# Autodesk Inventor assembly: Gripper V 10.0 assembly
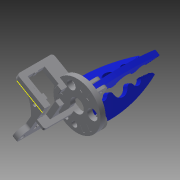
[picture p0: Inventor's stored thumbnail of the model, 180x180]
Saved by Autodesk Inventor 2015 (Build 190159000, 159)
## iProperties
Created: 2015-06-30
Part Number: Gripper V 10.0 assembly
Document SubType Name: Assembly
Designer: Stackpole
Author: Stackpole
## Documents named in this file (8)
- C:\Users\Stackpole\Desktop\Patrick!\Gripper Folder\Gripper V 10.0\Gripper V 10.0 assembly.iam
- C:\Users\Stackpole\Desktop\Patrick!\Gripper Folder\Gripper V 10.0\Gripper V 10.0 base 6mm.ipt
- C:\Users\Stackpole\Desktop\Patrick!\Gripper Folder\Gripper V 10.0\Gripper V 10.0 servo bracket right 6mm.ipt
- C:\Users\Stackpole\Desktop\Patrick!\Gripper Folder\Gripper V 10.0\Gripper V 10.1 servo bracket bottom 6mm.ipt
- C:\Users\Stackpole\Desktop\Patrick!\Gripper Folder\Gripper V 10.0\Gripper V 10.0 servo bracket side left 3mm.ipt
- C:\Users\Stackpole\Desktop\Patrick!\Gripper Folder\Gripper V 10.0\Gripper V 10.0 servo triangle bracket 3mm.ipt
- C:\Users\Stackpole\Desktop\Patrick!\Gripper Folder\Gripper V 10.0\Gripper V 10.0 base tab 3mm.ipt
- C:\Users\Stackpole\Desktop\Patrick!\Gripper Folder\Gripper V 10.0\Gripper V 10.0 finger master 6mm.ipt
## Components (14 placed, 7 different names)
1. Gripper V 10.0 base 6mm:1 — Mate:1, Mate:2, Mate:3, Mate:4, Mate:5, Mate:6, Mate:7, Mate:8, Mate:9, Mate:13, Mate:14, Mate:15, Mate:16, Mate:17, Mate:18, Mate:19, Mate:20, Mate:21, Mate:22, Mate:23, Mate:24, Mate:25, Mate:26, Mate:27, Mate:28, Mate:29, Mate:30, Mate:31
2. Gripper V 10.0 servo bracket right 6mm:1 — Mate:1, Mate:2, Mate:3, Mate:11
3. Gripper V 10.1 servo bracket bottom 6mm:1 — Mate:4, Mate:5, Mate:6, Mate:10, Mate:12
4. Gripper V 10.0 servo bracket side left 3mm:1 — Mate:7, Mate:8, Mate:9
5. Gripper V 10.0 servo triangle bracket 3mm:1 — Mate:10, Mate:11, Mate:12
6. Gripper V 10.0 finger master 6mm:1 — Insert:2
7. Gripper V 10.0 finger master 6mm:2 — Insert:3
8. Gripper V 10.0 finger master 6mm:3 — Insert:1
9. Gripper V 10.0 base tab 3mm:3 — Mate:13, Mate:22, Mate:27
10. Gripper V 10.0 base tab 3mm:4 — Mate:16, Mate:19, Mate:24, Mate:29
11. Gripper V 10.0 base tab 3mm:5 — Mate:17, Mate:20, Mate:31
12. Gripper V 10.0 base tab 3mm:6 — Mate:15, Mate:21, Mate:30, Insert:1
13. Gripper V 10.0 base tab 3mm:7 — Mate:14, Mate:25, Mate:28, Insert:2
14. Gripper V 10.0 base tab 3mm:8 — Mate:18, Mate:23, Mate:26, Insert:3
## Relationships (34: Mate 31, Insert 3)
- Mate:1: Gripper V 10.0 base 6mm:1 ↔ Gripper V 10.0 servo bracket right 6mm:1
- Mate:2: Gripper V 10.0 base 6mm:1 ↔ Gripper V 10.0 servo bracket right 6mm:1
- Mate:3: Gripper V 10.0 base 6mm:1 ↔ Gripper V 10.0 servo bracket right 6mm:1
- Mate:4: Gripper V 10.0 base 6mm:1 ↔ Gripper V 10.1 servo bracket bottom 6mm:1
- Mate:5: Gripper V 10.0 base 6mm:1 ↔ Gripper V 10.1 servo bracket bottom 6mm:1
- Mate:6: Gripper V 10.0 base 6mm:1 ↔ Gripper V 10.1 servo bracket bottom 6mm:1
- Mate:7: Gripper V 10.0 base 6mm:1 ↔ Gripper V 10.0 servo bracket side left 3mm:1
- Mate:8: Gripper V 10.0 base 6mm:1 ↔ Gripper V 10.0 servo bracket side left 3mm:1
- Mate:9: Gripper V 10.0 base 6mm:1 ↔ Gripper V 10.0 servo bracket side left 3mm:1
- Mate:10: Gripper V 10.1 servo bracket bottom 6mm:1 ↔ Gripper V 10.0 servo triangle bracket 3mm:1
- Mate:11: Gripper V 10.0 servo bracket right 6mm:1 ↔ Gripper V 10.0 servo triangle bracket 3mm:1
- Mate:12: Gripper V 10.1 servo bracket bottom 6mm:1 ↔ Gripper V 10.0 servo triangle bracket 3mm:1
- Mate:13: Gripper V 10.0 base 6mm:1 ↔ Gripper V 10.0 base tab 3mm:3
- Mate:14: Gripper V 10.0 base 6mm:1 ↔ Gripper V 10.0 base tab 3mm:7
- Mate:15: Gripper V 10.0 base 6mm:1 ↔ Gripper V 10.0 base tab 3mm:6
- Mate:16: Gripper V 10.0 base 6mm:1 ↔ Gripper V 10.0 base tab 3mm:4
- Mate:17: Gripper V 10.0 base 6mm:1 ↔ Gripper V 10.0 base tab 3mm:5
- Mate:18: Gripper V 10.0 base 6mm:1 ↔ Gripper V 10.0 base tab 3mm:8
- Mate:19: Gripper V 10.0 base 6mm:1 ↔ Gripper V 10.0 base tab 3mm:4
- Mate:20: Gripper V 10.0 base 6mm:1 ↔ Gripper V 10.0 base tab 3mm:5
- Mate:21: Gripper V 10.0 base 6mm:1 ↔ Gripper V 10.0 base tab 3mm:6
- Mate:22: Gripper V 10.0 base 6mm:1 ↔ Gripper V 10.0 base tab 3mm:3
- Mate:23: Gripper V 10.0 base 6mm:1 ↔ Gripper V 10.0 base tab 3mm:8
- Mate:24: Gripper V 10.0 base 6mm:1 ↔ Gripper V 10.0 base tab 3mm:4
- Mate:25: Gripper V 10.0 base 6mm:1 ↔ Gripper V 10.0 base tab 3mm:7
- Mate:26: Gripper V 10.0 base 6mm:1 ↔ Gripper V 10.0 base tab 3mm:8
- Mate:27: Gripper V 10.0 base 6mm:1 ↔ Gripper V 10.0 base tab 3mm:3
- Mate:28: Gripper V 10.0 base 6mm:1 ↔ Gripper V 10.0 base tab 3mm:7
- Mate:29: Gripper V 10.0 base 6mm:1 ↔ Gripper V 10.0 base tab 3mm:4
- Mate:30: Gripper V 10.0 base 6mm:1 ↔ Gripper V 10.0 base tab 3mm:6
- Mate:31: Gripper V 10.0 base 6mm:1 ↔ Gripper V 10.0 base tab 3mm:5
- Insert:1: Gripper V 10.0 finger master 6mm:3 ↔ Gripper V 10.0 base tab 3mm:6
- Insert:2: Gripper V 10.0 finger master 6mm:1 ↔ Gripper V 10.0 base tab 3mm:7
- Insert:3: Gripper V 10.0 finger master 6mm:2 ↔ Gripper V 10.0 base tab 3mm:8
